# Autodesk Inventor assembly: mr-20cnb_mrs20-1200_0_MIR
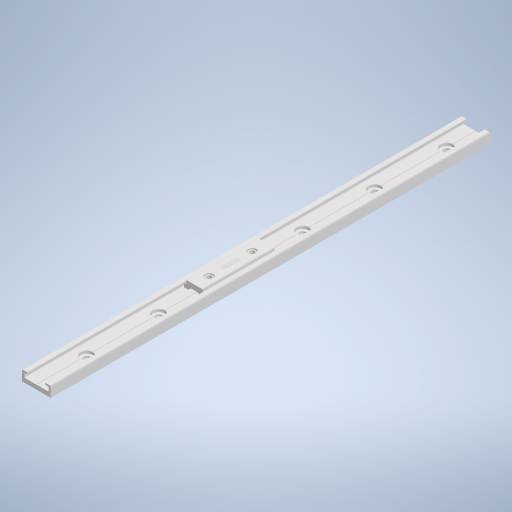
[picture p0: Inventor's stored thumbnail of the model, 512x512]
Saved by Autodesk Inventor 2024.1 (Build 281209000, 209)
## iProperties
Created: 2020-09-01
Part Number: mr-20cnb_mrs20-1200_0_MIR
Description: STEP AP203
Document SubType Name: Assembly
Designer: haruy
Sending System: SolidWorks 2017
Preprocessor: SwSTEP 2.0
Title: MR-20CNB_MRS20-1200_0.step
Revision Number: ANY
## Documents named in this file (3)
- C:\Users\haruy\OneDrive - Kyushu University\KURT_工房共有\2023~2024\ハード\CAD\2024NHK\000_parts\スライダー\mr-20cnb_mrs20-1200_0_MIR.iam
- C:\Users\haruy\OneDrive - Kyushu University\KURT_工房共有\2023~2024\ハード\CAD\2024NHK\000_parts\スライダー\MR-20CNB_MIR.iam
- C:\Users\haruy\OneDrive - Kyushu University\KURT_工房共有\2023~2024\ハード\CAD\2024NHK\000_parts\スライダー\mrs20-1200_MIR.ipt
## Components (2 placed, 2 different names)
1. MR-20CNB_MIR:1 [sub-assembly] — メイト:3, メイト:2, メイト:1
2. mrs20-1200_MIR:1 — メイト:3, メイト:2, メイト:1
## Relationships (3: Mate 3)
- メイト:3 [Mate] (0.1 mm): MR-20CNB_MIR:1 ↔ mrs20-1200_MIR:1
- メイト:2 [Mate] (0.1 mm): MR-20CNB_MIR:1 ↔ mrs20-1200_MIR:1
- メイト:1 [Mate]: MR-20CNB_MIR:1 ↔ mrs20-1200_MIR:1
